# Autodesk Inventor assembly: FP Assembly Race Car
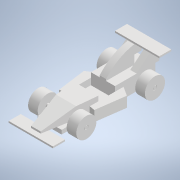
[picture p0: Inventor's stored thumbnail of the model, 180x180]
Saved by Autodesk Inventor 2020 (Build 240168000, 168)
## iProperties
Created: 2021-05-05
Part Number: FP Assembly Race Car
Document SubType Name: Assembly
Designer: austi
Author: austi
## Documents named in this file (10)
- D:\Final Project\FP Assembly Race Car.iam
- D:\Final Project\FP Axle (2).ipt
- D:\Final Project\FP Chassis.ipt
- D:\Final Project\FP Cockpit.ipt
- D:\Final Project\FP Front Hood.ipt
- D:\Final Project\FP Rear Hood.ipt
- D:\Final Project\FP Side Boards (2).ipt
- D:\Final Project\FP Spoilers (2).ipt
- D:\Final Project\FP Struts (2).ipt
- D:\Final Project\FP Wheel (4).ipt
## Components (16 placed, 9 different names)
1. FP Axle (2):1 — Mate:9, Flush:8, Mate:12, Flush:9, Tangent:3, Tangent:4
2. FP Chassis:1 — Mate:1, Flush:1, Angle:1, Angle:2, Mate:2, Angle:3, Angle:4, Mate:3, Mate:4, Mate:5, Flush:2, Flush:3, Mate:6, Mate:7, Angle:5, Angle:7, Mate:8, Flush:4, Flush:5, Flush:6, Flush:12, Angle:15, Angle:16, Angle:17, Angle:18, Angle:19, Tangent:1, Tangent:3
3. FP Cockpit:1 — Angle:17, Angle:18, Angle:19, Flush:17, Mate:17, Flush:18
4. FP Front Hood:1 — Angle:1, Angle:2, Mate:2, Mate:4, Mate:5, Flush:2, Angle:6, Angle:8, Angle:9, Mate:13, Flush:11, Tangent:4
5. FP Rear Hood:1 — Angle:5, Angle:6, Angle:7, Mate:8, Flush:4, Flush:5, Flush:6, Mate:15, Flush:13, Flush:14, Flush:15, Mate:16, Flush:17, Mate:17, Flush:18, Tangent:2
6. FP Side Boards (2):1 — Angle:3, Angle:4, Mate:3, Flush:3, Mate:6
7. FP Spoilers (2):1 — Angle:8, Mate:14, Angle:13, Angle:14, Flush:19, Flush:20
8. FP Struts (2):1 — Angle:12, Flush:15, Mate:16, Flush:16
9. FP Wheel (4):1 — Mate:9, Flush:8, Angle:16, Flush:21
10. FP Axle (2):2 — Mate:10, Flush:7, Mate:11, Flush:10, Tangent:1, Tangent:2
11. FP Side Boards (2):2 — Mate:1, Flush:1, Mate:7
12. FP Spoilers (2):2 — Angle:9, Mate:13, Flush:11, Flush:12, Flush:19, Flush:21, Flush:22
13. FP Struts (2):2 — Angle:12, Mate:14, Angle:13, Angle:14, Mate:15, Flush:13, Flush:14, Flush:16, Flush:20
14. FP Wheel (4):2 — Mate:10, Flush:7, Angle:15, Flush:22
15. FP Wheel (4):3 — Mate:12, Flush:9
16. FP Wheel (4):4 — Mate:11, Flush:10
## Relationships (60: Flush 22, Mate 17, Angle 17, Tangent 4)
- Mate:1: FP Chassis:1 ↔ FP Side Boards (2):2
- Flush:1: FP Chassis:1 ↔ FP Side Boards (2):2
- Angle:1 (0 deg): FP Chassis:1 ↔ FP Front Hood:1
- Angle:2 (0 deg): FP Chassis:1 ↔ FP Front Hood:1
- Mate:2: FP Chassis:1 ↔ FP Front Hood:1
- Angle:3 (0 deg): FP Chassis:1 ↔ FP Side Boards (2):1
- Angle:4 (0 deg): FP Chassis:1 ↔ FP Side Boards (2):1
- Mate:3: FP Chassis:1 ↔ FP Side Boards (2):1
- Mate:4: FP Chassis:1 ↔ FP Front Hood:1
- Mate:5: FP Chassis:1 ↔ FP Front Hood:1
- Flush:2 (18.034 mm): FP Chassis:1 ↔ FP Front Hood:1
- Flush:3: FP Chassis:1 ↔ FP Side Boards (2):1
- Mate:6 (33.02 mm): FP Chassis:1 ↔ FP Side Boards (2):1
- Mate:7 (33.02 mm): FP Chassis:1 ↔ FP Side Boards (2):2
- Angle:5 (0 deg): FP Chassis:1 ↔ FP Rear Hood:1
- Angle:6 (0 deg): FP Front Hood:1 ↔ FP Rear Hood:1
- Angle:7 (0 deg): FP Chassis:1 ↔ FP Rear Hood:1
- Mate:8: FP Chassis:1 ↔ FP Rear Hood:1
- Flush:4: FP Chassis:1 ↔ FP Rear Hood:1
- Flush:5: FP Chassis:1 ↔ FP Rear Hood:1
- Flush:6 (6.35 mm): FP Chassis:1 ↔ FP Rear Hood:1
- Mate:9: FP Axle (2):1 ↔ FP Wheel (4):1
- Mate:10: FP Axle (2):2 ↔ FP Wheel (4):2
- Flush:7: FP Axle (2):2 ↔ FP Wheel (4):2
- Flush:8: FP Axle (2):1 ↔ FP Wheel (4):1
- Mate:11: FP Axle (2):2 ↔ FP Wheel (4):4
- Mate:12: FP Axle (2):1 ↔ FP Wheel (4):3
- Flush:9: FP Axle (2):1 ↔ FP Wheel (4):3
- Flush:10: FP Axle (2):2 ↔ FP Wheel (4):4
- Angle:8 (0 deg): FP Front Hood:1 ↔ FP Spoilers (2):1
- Angle:9 (0 deg): FP Front Hood:1 ↔ FP Spoilers (2):2
- Mate:13: FP Front Hood:1 ↔ FP Spoilers (2):2
- Flush:11 (6.35 mm): FP Front Hood:1 ↔ FP Spoilers (2):2
- Flush:12 (12.446 mm): FP Chassis:1 ↔ FP Spoilers (2):2
- Angle:12 (0 deg): FP Struts (2):1 ↔ FP Struts (2):2
- Mate:14: FP Spoilers (2):1 ↔ FP Struts (2):2
- Angle:13 (0 deg): FP Spoilers (2):1 ↔ FP Struts (2):2
- Angle:14 (0 deg): FP Spoilers (2):1 ↔ FP Struts (2):2
- Mate:15: FP Rear Hood:1 ↔ FP Struts (2):2
- Flush:13: FP Rear Hood:1 ↔ FP Struts (2):2
- Flush:14 (5 mm): FP Rear Hood:1 ↔ FP Struts (2):2
- Angle:15 (0 deg): FP Chassis:1 ↔ FP Wheel (4):2
- Angle:16 (0 deg): FP Chassis:1 ↔ FP Wheel (4):1
- Flush:15: FP Rear Hood:1 ↔ FP Struts (2):1
- Mate:16: FP Rear Hood:1 ↔ FP Struts (2):1
- Flush:16: FP Struts (2):1 ↔ FP Struts (2):2
- Angle:17 (0 deg): FP Chassis:1 ↔ FP Cockpit:1
- Angle:18 (0 deg): FP Chassis:1 ↔ FP Cockpit:1
- Angle:19 (0 deg): FP Chassis:1 ↔ FP Cockpit:1
- Flush:17: FP Cockpit:1 ↔ FP Rear Hood:1
- Mate:17: FP Cockpit:1 ↔ FP Rear Hood:1
- Flush:18 (10.922 mm): FP Cockpit:1 ↔ FP Rear Hood:1
- Tangent:1: FP Chassis:1 ↔ FP Axle (2):2
- Tangent:2: FP Rear Hood:1 ↔ FP Axle (2):2
- Tangent:3: FP Axle (2):1 ↔ FP Chassis:1
- Tangent:4: FP Axle (2):1 ↔ FP Front Hood:1
- Flush:19: FP Spoilers (2):1 ↔ FP Spoilers (2):2
- Flush:20 (2.54 mm): FP Spoilers (2):1 ↔ FP Struts (2):2
- Flush:21 (-2.54 mm): FP Wheel (4):1 ↔ FP Spoilers (2):2
- Flush:22 (-2.54 mm): FP Spoilers (2):2 ↔ FP Wheel (4):2
